# Autodesk Inventor assembly: QuadCopter
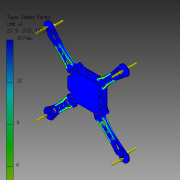
[picture p0: Inventor's stored thumbnail of the model, 180x180]
Saved by Autodesk Inventor 2015 (Build 190159000, 159)
## iProperties
Created: 2015-06-01
Part Number: QuadCopter
Document SubType Name: Assembly
Designer: Vu
Mass: 335.672 g
Surface Area: 1572.18 cm^2
Volume: 316.671 cm^3
Density: 1.06 g/cm^3
Author: Vu
## Documents named in this file (10)
- C:\Users\Vu\Documents\QuadCopter\models\heavyRevision\QuadCopter.iam
- C:\Users\Vu\Documents\QuadCopter\models\heavyRevision\LowerPlatter.ipt
- C:\Users\Vu\Documents\QuadCopter\models\heavyRevision\Arm.ipt
- C:\Users\Vu\Documents\QuadCopter\models\heavyRevision\Ceiling.ipt
- C:\Users\Vu\Documents\QuadCopter\models\heavyRevision\QuadCopter\AIP\FEA\bjrzdrf9c.fins
- C:\Users\Vu\Documents\QuadCopter\models\heavyRevision\QuadCopter\AIP\FEA\bjrzdrfeo.fsat
- C:\Users\Vu\Documents\QuadCopter\models\heavyRevision\QuadCopter\AIP\FEA\bjrzdrfj4.ftes
- C:\Users\Vu\Documents\QuadCopter\models\heavyRevision\QuadCopter\AIP\FEA\bjrzdrfnk.fwiz
- C:\Users\Vu\Documents\QuadCopter\models\heavyRevision\QuadCopter\AIP\FEA\bjs1y38io.fmsh
- C:\Users\Vu\Documents\QuadCopter\models\heavyRevision\QuadCopter\AIP\FEA\bjs1y38kg.fres
## Components (6 placed, 3 different names)
1. LowerPlatter:1 — Mate:1, Mate:2, Mate:3, Mate:4, Mate:5, Mate:6, Mate:7, Mate:8, Mate:9, Mate:10, Mate:11, Mate:12
2. Arm:1 — Mate:1, Mate:2, Mate:3, Mate:13
3. Arm:2 — Mate:4, Mate:5, Mate:6
4. Arm:3 — Mate:10, Mate:11, Mate:12
5. Arm:4 — Mate:7, Mate:8, Mate:9, Mate:14, Mate:15
6. Ceiling:1 — Mate:13, Mate:14, Mate:15
## Relationships (15: Mate 15)
- Mate:1: LowerPlatter:1 ↔ Arm:1
- Mate:2: LowerPlatter:1 ↔ Arm:1
- Mate:3: LowerPlatter:1 ↔ Arm:1
- Mate:4: LowerPlatter:1 ↔ Arm:2
- Mate:5: LowerPlatter:1 ↔ Arm:2
- Mate:6: LowerPlatter:1 ↔ Arm:2
- Mate:7: LowerPlatter:1 ↔ Arm:4
- Mate:8: LowerPlatter:1 ↔ Arm:4
- Mate:9: LowerPlatter:1 ↔ Arm:4
- Mate:10: LowerPlatter:1 ↔ Arm:3
- Mate:11: LowerPlatter:1 ↔ Arm:3
- Mate:12: LowerPlatter:1 ↔ Arm:3
- Mate:13: Arm:1 ↔ Ceiling:1
- Mate:14: Arm:4 ↔ Ceiling:1
- Mate:15: Arm:4 ↔ Ceiling:1
## Named parameters: sa_1 = 0, sa_2 = 784.8, sa_3 = 0, sa_0 = 0, sa_4 = 784.8, sa_5 = -1e-13, sa_6 = 0, sa_7 = 784.8, sa_8 = 0, sa_9 = 0, sa_10 = 784.8, sa_11 = 0, sa_12 = 0, sa_13 = -98.1, sa_14 = 0, sa_15 = 0, sa_16 = -981, sa_17 = 0, sa_18 = -2e-13, sa_19 = -500, sa_20 = 2e-13
note: some values were not read from the file. Shown as the stored number, unit unknown: "sa_1", "sa_2", "sa_3", "sa_0", "sa_4", "sa_5", "sa_6", "sa_7", "sa_8", "sa_9", "sa_10", "sa_11", "sa_12", "sa_13", "sa_14", "sa_15", "sa_16", "sa_17", "sa_18", "sa_19", "sa_20".
